# Autodesk Inventor assembly: Chasis Montaje 2m
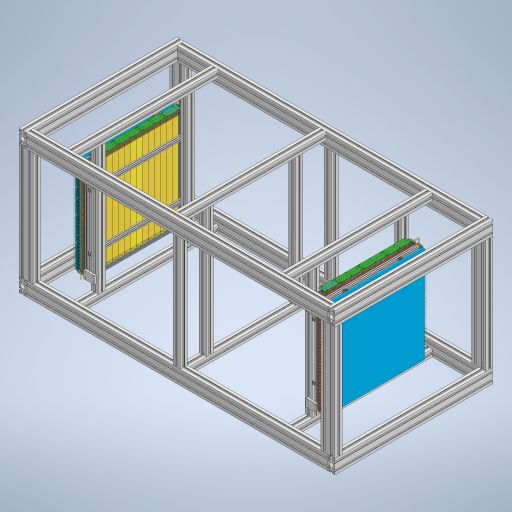
[picture p0: Inventor's stored thumbnail of the model, 512x512]
Saved by Autodesk Inventor 2024.2 (Build 282272000, 272)
## iProperties
Created: 2025-06-05
Part Number: Chasis Montaje 2m
Document SubType Name: Assembly
Designer: ja.restrepo1
Author: ja.restrepo1
## Documents named in this file (6)
- I:\MICROMECANICA\ALTAS ENERGIAS\Deteccion de Muones\Detectores centelladores\Partes Detectores centelladores\Chasis DC\Chasis Montaje 2m.iam
- I:\MICROMECANICA\ALTAS ENERGIAS\Deteccion de Muones\Detectores centelladores\Partes Detectores centelladores\PARTES DC\EG Detector Centellador.iam
- I:\MICROMECANICA\ALTAS ENERGIAS\Deteccion de Muones\Detectores centelladores\Partes Detectores centelladores\Chasis DC\Partes Chasis DC\Soporte.ipt
- I:\MICROMECANICA\ALTAS ENERGIAS\Deteccion de Muones\Detectores centelladores\Partes Detectores centelladores\Chasis DC\Partes Chasis DC\Lamina centelladora.ipt
- I:\MICROMECANICA\ALTAS ENERGIAS\Deteccion de Muones\Detectores centelladores\Partes Detectores centelladores\Chasis DC\Partes Chasis DC\Sujecion centelladora.iam
- I:\MICROMECANICA\ALTAS ENERGIAS\Deteccion de Muones\Detectores centelladores\Partes Detectores centelladores\Chasis DC\SE. Chasis DC 2m.iam
## Components (17 placed, 5 different names)
1. SE. Chasis DC 2m:1 [sub-assembly] — Nivelación:1, Nivelación:2, Nivelación:3, Coincidencia:1, Ángulo:1, Ángulo:2, Coincidencia:5, Coincidencia:6, Coincidencia:7, Nivelación:7, Coincidencia:10, Coincidencia:12, Coincidencia:14, Coincidencia:16, Coincidencia:24, Coincidencia:25, Coincidencia:26, Coincidencia:27, Coincidencia:28, Coincidencia:29, Coincidencia:30, Coincidencia:31
2. EG Detector Centellador:1 [sub-assembly] — Ángulo:1, Coincidencia:5, Nivelación:5, Nivelación:6, Coincidencia:6, Coincidencia:40, Nivelación:22, Coincidencia:41
3. EG Detector Centellador:2 [sub-assembly] — Ángulo:2, Nivelación:5, Nivelación:6, Coincidencia:7, Nivelación:7, Coincidencia:8, Coincidencia:9, Coincidencia:11, Nivelación:8, Coincidencia:13, Coincidencia:15, Coincidencia:23, Nivelación:16, Nivelación:17, Coincidencia:42, Coincidencia:43, Coincidencia:44, Coincidencia:45, Coincidencia:46, Coincidencia:47, Coincidencia:48, Coincidencia:49, Coincidencia:50, Coincidencia:51, Coincidencia:52, Coincidencia:53
4. Soporte:1 — Coincidencia:8, Coincidencia:9, Coincidencia:12, Nivelación:10, Nivelación:12
5. Soporte:2 — Coincidencia:10, Coincidencia:11, Nivelación:8, Nivelación:9, Nivelación:13
6. Soporte:3 — Coincidencia:13, Coincidencia:14, Nivelación:9, Nivelación:15
7. Soporte:4 — Coincidencia:15, Coincidencia:16, Nivelación:10, Nivelación:14
8. Lamina centelladora:1 — Coincidencia:23, Nivelación:16, Nivelación:17
9. Soporte:5 — Coincidencia:26, Coincidencia:27, Nivelación:13
10. Soporte:6 — Coincidencia:24, Coincidencia:25, Nivelación:12
11. Soporte:7 — Coincidencia:28, Coincidencia:29, Nivelación:14
12. Soporte:8 — Coincidencia:30, Coincidencia:31, Nivelación:15
13. Lamina centelladora:2 — Coincidencia:40, Nivelación:22, Coincidencia:41
14. Sujecion centelladora:1 [sub-assembly] — Coincidencia:42, Coincidencia:43, Coincidencia:44
15. Sujecion centelladora:2 [sub-assembly] — Coincidencia:48, Coincidencia:49, Coincidencia:50
16. Sujecion centelladora:4 [sub-assembly] — Coincidencia:45, Coincidencia:46, Coincidencia:47
17. Sujecion centelladora:6 [sub-assembly] — Coincidencia:51, Coincidencia:52, Coincidencia:53
## Relationships (54: Mate 36, Flush 16, Angle 2)
- Nivelación:1 [Flush]: SE. Chasis DC 2m:1
- Nivelación:2 [Flush]: SE. Chasis DC 2m:1
- Nivelación:3 [Flush]: SE. Chasis DC 2m:1
- Coincidencia:1 [Mate]: SE. Chasis DC 2m:1
- Ángulo:1 [Angle] (0 deg): SE. Chasis DC 2m:1 ↔ EG Detector Centellador:1
- Ángulo:2 [Angle] (0 deg): SE. Chasis DC 2m:1 ↔ EG Detector Centellador:2
- Coincidencia:5 [Mate] (10 mm): SE. Chasis DC 2m:1 ↔ EG Detector Centellador:1
- Nivelación:5 [Flush]: EG Detector Centellador:1 ↔ EG Detector Centellador:2
- Nivelación:6 [Flush]: EG Detector Centellador:1 ↔ EG Detector Centellador:2
- Coincidencia:6 [Mate]: SE. Chasis DC 2m:1 ↔ EG Detector Centellador:1
- Coincidencia:7 [Mate]: SE. Chasis DC 2m:1 ↔ EG Detector Centellador:2
- Nivelación:7 [Flush]: SE. Chasis DC 2m:1 ↔ EG Detector Centellador:2
- Coincidencia:8 [Mate]: EG Detector Centellador:2 ↔ Soporte:1
- Coincidencia:9 [Mate]: EG Detector Centellador:2 ↔ Soporte:1
- Coincidencia:10 [Mate]: SE. Chasis DC 2m:1 ↔ Soporte:2
- Coincidencia:11 [Mate]: EG Detector Centellador:2 ↔ Soporte:2
- Coincidencia:12 [Mate] (50 mm): SE. Chasis DC 2m:1 ↔ Soporte:1
- Nivelación:8 [Flush] (50 mm): EG Detector Centellador:2 ↔ Soporte:2
- Coincidencia:13 [Mate]: EG Detector Centellador:2 ↔ Soporte:3
- Coincidencia:14 [Mate]: SE. Chasis DC 2m:1 ↔ Soporte:3
- Nivelación:9 [Flush]: Soporte:2 ↔ Soporte:3
- Coincidencia:15 [Mate]: EG Detector Centellador:2 ↔ Soporte:4
- Coincidencia:16 [Mate]: SE. Chasis DC 2m:1 ↔ Soporte:4
- Nivelación:10 [Flush]: Soporte:1 ↔ Soporte:4
- Coincidencia:23 [Mate]: EG Detector Centellador:2 ↔ Lamina centelladora:1
- Coincidencia:24 [Mate]: SE. Chasis DC 2m:1 ↔ Soporte:6
- Coincidencia:25 [Mate]: SE. Chasis DC 2m:1 ↔ Soporte:6
- Nivelación:12 [Flush]: Soporte:1 ↔ Soporte:6
- Coincidencia:26 [Mate]: SE. Chasis DC 2m:1 ↔ Soporte:5
- Coincidencia:27 [Mate]: SE. Chasis DC 2m:1 ↔ Soporte:5
- Nivelación:13 [Flush]: Soporte:2 ↔ Soporte:5
- Coincidencia:28 [Mate]: SE. Chasis DC 2m:1 ↔ Soporte:7
- Coincidencia:29 [Mate]: SE. Chasis DC 2m:1 ↔ Soporte:7
- Nivelación:14 [Flush]: Soporte:4 ↔ Soporte:7
- Coincidencia:30 [Mate]: SE. Chasis DC 2m:1 ↔ Soporte:8
- Coincidencia:31 [Mate]: SE. Chasis DC 2m:1 ↔ Soporte:8
- Nivelación:15 [Flush]: Soporte:3 ↔ Soporte:8
- Nivelación:16 [Flush]: EG Detector Centellador:2 ↔ Lamina centelladora:1
- Nivelación:17 [Flush]: EG Detector Centellador:2 ↔ Lamina centelladora:1
- Coincidencia:40 [Mate]: EG Detector Centellador:1 ↔ Lamina centelladora:2
- Nivelación:22 [Flush]: EG Detector Centellador:1 ↔ Lamina centelladora:2
- Coincidencia:41 [Mate]: EG Detector Centellador:1 ↔ Lamina centelladora:2
- Coincidencia:42 [Mate]: EG Detector Centellador:2 ↔ Sujecion centelladora:1
- Coincidencia:43 [Mate]: EG Detector Centellador:2 ↔ Sujecion centelladora:1
- Coincidencia:44 [Mate]: EG Detector Centellador:2 ↔ Sujecion centelladora:1
- Coincidencia:45 [Mate]: EG Detector Centellador:2 ↔ Sujecion centelladora:4
- Coincidencia:46 [Mate]: EG Detector Centellador:2 ↔ Sujecion centelladora:4
- Coincidencia:47 [Mate]: EG Detector Centellador:2 ↔ Sujecion centelladora:4
- Coincidencia:48 [Mate]: EG Detector Centellador:2 ↔ Sujecion centelladora:2
- Coincidencia:49 [Mate]: EG Detector Centellador:2 ↔ Sujecion centelladora:2
- Coincidencia:50 [Mate]: EG Detector Centellador:2 ↔ Sujecion centelladora:2
- Coincidencia:51 [Mate]: EG Detector Centellador:2 ↔ Sujecion centelladora:6
- Coincidencia:52 [Mate]: EG Detector Centellador:2 ↔ Sujecion centelladora:6
- Coincidencia:53 [Mate]: EG Detector Centellador:2 ↔ Sujecion centelladora:6
